# Autodesk Inventor assembly: Assy_wrist
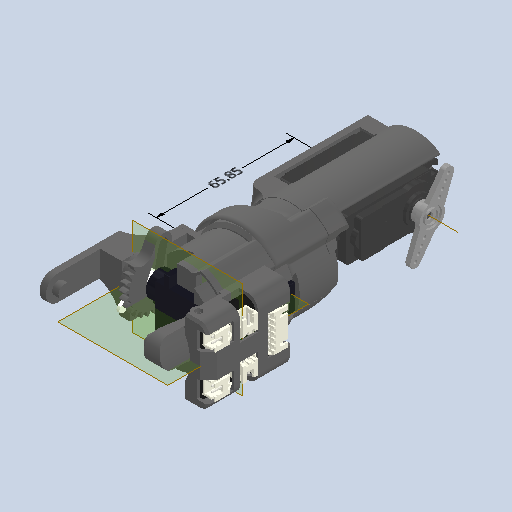
[picture p0: Inventor's stored thumbnail of the model, 512x512]
Saved by Autodesk Inventor 2024.1 (Build 281209000, 209)
## iProperties
Created: 2025-03-02
Part Number: Assy_wrist
Document SubType Name: Assembly
Designer: hibik
Author: hibik
## Documents named in this file (3)
- C:\Users\hibik\Documents\Robomech\RESCUE\ORCA\hard\arm\Assy_wrist.iam
- C:\Users\hibik\Documents\Robomech\RESCUE\ORCA\hard\arm\Assy_wrist_back.iam
- C:\Users\hibik\Documents\Robomech\RESCUE\ORCA\hard\arm\Assy_wrist_fore.iam
## Components (2 placed, 2 different names)
1. Assy_wrist_back:1 [sub-assembly] — 挿入:1
2. Assy_wrist_fore:1 [sub-assembly] — 挿入:1
## Relationships (1: Insert 1)
- 挿入:1 [Insert] (0.5 mm): Assy_wrist_back:1 ↔ Assy_wrist_fore:1
